# Autodesk Inventor assembly: robot_no_arm
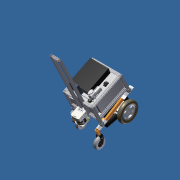
[picture p0: Inventor's stored thumbnail of the model, 180x180]
Saved by Autodesk Inventor 2012 (Build 160160000, 160)
## iProperties
Created: 2012-03-08
Part Number: robot_no_arm
Document SubType Name: Assembly
Designer: esv
Mass: 187059 g
Surface Area: 125343 cm^2
Volume: 160092 cm^3
Density: 1.16845 g/cm^3
Author: esv
## Documents named in this file (16)
- C:\Users\Ed\Documents\masters\CAD\robot_no_arm.iam
- C:\Users\Ed\Documents\masters\CAD\Frame\frame bracket.ipt
- C:\Users\Ed\Documents\masters\CAD\Invacare\invacare assy.iam
- C:\Users\Ed\Documents\masters\CAD\IRC5\IRC5_Compact.ipt
- C:\Users\Ed\Documents\masters\CAD\PC\PC.ipt
- C:\Users\Ed\Documents\masters\CAD\SICK\SICK LMS291.ipt
- C:\Users\Ed\Documents\masters\CAD\Frame\back frame plate.ipt
- C:\Users\Ed\Documents\masters\CAD\Frame\front frame plate.ipt
- C:\Users\Ed\Documents\masters\CAD\Frame\top plate.ipt
- C:\Users\Ed\Documents\masters\CAD\Pneumatics\compressor\compressor.iam
- C:\Users\Ed\Documents\masters\CAD\Spike\Spike H.iam
- C:\Users\Ed\Documents\masters\CAD\Breaker\Breaker.iam
- C:\Users\Ed\Documents\masters\CAD\Router\router keepout.ipt
- C:\Users\Ed\Documents\masters\CAD\Frame\short frame bracket.ipt
- C:\Users\Ed\Documents\masters\CAD\base plate.iam
- C:\Users\Ed\Documents\masters\CAD\al_frame.iam
## Components (19 placed, 19 different names)
1. f_r_frame_bracket — Flush:5, Mate:72, Flush:56, Mate:74, Mate:132
2. f_l_frame_bracket — Flush:5, Flush:57, Mate:75, Mate:76
3. drive_base [sub-assembly] — Mate:17, Flush:96, Tangent:8, Mate:97
4. IRC5_Compact — Flush:2, Mate:122, Mate:126
5. PC — Mate:36, Flush:63, Flush:91
6. SICK_LMS291 — Mate:118, Insert:12
7. b_l_frame_plate — Flush:82, Insert:7, Flush:88, Flush:89, Flush:96, Tangent:8, Flush:98
8. b_r_frame_plate — Insert:6, Flush:87, Flush:88, Flush:90, Flush:100
9. f_l_frame_plate — Flush:57, Mate:75, Mate:76, Flush:89, Mate:97, Flush:98, Flush:99
10. f_r_frame_plate — Mate:72, Flush:56, Mate:74, Flush:90, Flush:99, Flush:100
11. top_plate — Mate:36, Mate:80, Flush:63, Mate:81, Insert:1, Insert:2, Insert:3, Mate:82, Insert:4, Insert:5, Flush:64, Mate:121, Flush:85, Flush:86, Flush:91
12. compressor [sub-assembly] — Mate:80, Insert:2, Insert:3
13. spike_relay [sub-assembly] — Mate:81, Insert:1
14. main_breaker [sub-assembly] — Mate:82, Insert:4, Insert:5
15. router — Flush:64, Mate:83, Mate:119
16. b_r_frame_bracket — Insert:6, Flush:87, Mate:127, Mate:129, Mate:130
17. b_l_frame_bracket — Flush:82, Insert:7, Mate:131
18. base_plate [sub-assembly] — Mate:123, Mate:124, Mate:125, Mate:126
19. frame [sub-assembly] — Mate:119, Mate:121, Flush:85, Flush:86, Mate:122, Insert:12, Mate:123, Mate:124, Mate:125, Mate:127, Mate:129, Mate:130, Mate:131, Mate:132
## Relationships (53: Mate 25, Flush 19, Insert 8, Tangent 1)
- Flush:2 (-225 mm): IRC5_Compact
- Flush:5: f_r_frame_bracket ↔ f_l_frame_bracket
- Mate:17: drive_base
- Mate:36: PC ↔ top_plate
- Flush:40 (-368.3 mm)
- Mate:56
- Mate:72: f_r_frame_bracket ↔ f_r_frame_plate
- Flush:56: f_r_frame_bracket ↔ f_r_frame_plate
- Mate:74: f_r_frame_bracket ↔ f_r_frame_plate
- Flush:57: f_l_frame_bracket ↔ f_l_frame_plate
- Mate:75: f_l_frame_bracket ↔ f_l_frame_plate
- Mate:76: f_l_frame_bracket ↔ f_l_frame_plate
- Mate:80: top_plate ↔ compressor
- Flush:63 (-50.8 mm): PC ↔ top_plate
- Mate:81: top_plate ↔ spike_relay
- Insert:1: top_plate ↔ spike_relay
- Insert:2: top_plate ↔ compressor
- Insert:3: top_plate ↔ compressor
- Mate:82: top_plate ↔ main_breaker
- Insert:4: top_plate ↔ main_breaker
- Insert:5: top_plate ↔ main_breaker
- Flush:64 (-304.8 mm): top_plate ↔ router
- Mate:83: router
- Insert:6: b_r_frame_plate ↔ b_r_frame_bracket
- Flush:82: b_l_frame_plate ↔ b_l_frame_bracket
- Insert:7: b_l_frame_plate ↔ b_l_frame_bracket
- Mate:118: SICK_LMS291
- Mate:119: router ↔ frame
- Mate:121: top_plate ↔ frame
- Flush:85: top_plate ↔ frame
- Flush:86: top_plate ↔ frame
- Mate:122: IRC5_Compact ↔ frame
- Insert:12: SICK_LMS291 ↔ frame
- Mate:123: base_plate ↔ frame
- Mate:124: base_plate ↔ frame
- Mate:125: base_plate ↔ frame
- Mate:126: IRC5_Compact ↔ base_plate
- Flush:87: b_r_frame_plate ↔ b_r_frame_bracket
- Flush:88: b_l_frame_plate ↔ b_r_frame_plate
- Flush:89: b_l_frame_plate ↔ f_l_frame_plate
- Flush:90: b_r_frame_plate ↔ f_r_frame_plate
- Mate:127: b_r_frame_bracket ↔ frame
- Mate:129: b_r_frame_bracket ↔ frame
- Mate:130: b_r_frame_bracket ↔ frame
- Mate:131: b_l_frame_bracket ↔ frame
- Flush:91 (50.8 mm): PC ↔ top_plate
- Mate:132: f_r_frame_bracket ↔ frame
- Flush:96 (88.9 mm): drive_base ↔ b_l_frame_plate
- Tangent:8: drive_base ↔ b_l_frame_plate
- Mate:97: drive_base ↔ f_l_frame_plate
- Flush:98: b_l_frame_plate ↔ f_l_frame_plate
- Flush:99: f_l_frame_plate ↔ f_r_frame_plate
- Flush:100: b_r_frame_plate ↔ f_r_frame_plate
